# Autodesk Inventor assembly: ユニット4
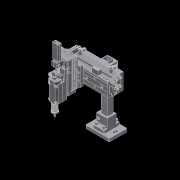
[picture p0: Inventor's stored thumbnail of the model, 180x180]
Saved by Autodesk Inventor 2021.1 (Build 251245010, 245A)
## iProperties
Created: 2008-11-13
Document SubType Name: Assembly
Title: ユニット4
## Documents named in this file (35)
- Z:\inventorroom\sample\unit4\unit4.iam
- Z:\inventorroom\sample\unit4\03.ipt
- Z:\inventorroom\sample\unit4\04.ipt
- Z:\inventorroom\sample\unit4\WSSM20-10-3.ipt
- Z:\inventorroom\sample\unit4\MHCAW10.ipt
- Z:\inventorroom\sample\unit4\07.ipt
- Z:\inventorroom\sample\unit4\AS1201F-M5-04.ipt
- Z:\inventorroom\sample\unit4\MXQ12-40AS\MXQ12-40AS-M9B.iam
- Z:\inventorroom\sample\unit4\MXQ16-75A\MXQ16-75A-M9B.iam
- Z:\inventorroom\sample\unit4\GT-H10.ipt
- Z:\inventorroom\sample\unit4\KJL06-M5.ipt
- Z:\inventorroom\sample\unit4\STAQ20-200.ipt
- Z:\inventorroom\sample\unit4\01.ipt
- Z:\inventorroom\sample\unit4\02.ipt
- Z:\inventorroom\sample\unit4\06.ipt
- Z:\inventorroom\sample\unit4\PSPWR10_100_M5_N6_SC10.ipt
- Z:\inventorroom\sample\unit4\SWU17_30.ipt
- Z:\inventorroom\sample\unit4\PSCKNK10-10\PSCKNK10-10.iam
- Z:\inventorroom\sample\unit4\05.ipt
- Z:\inventorroom\sample\unit4\CBM5_18.ipt
- Z:\inventorroom\sample\unit4\PWF5.ipt
- Z:\inventorroom\sample\unit4\SLW5.ipt
- Z:\inventorroom\sample\unit4\CLQAM20\CLQAM20.iam
- Z:\inventorroom\sample\unit4\CLTQAM20\CLTQAM20.iam
- Z:\inventorroom\sample\unit4\CBM5_30.ipt
- Z:\inventorroom\sample\unit4\CBM5_10.ipt
- Z:\inventorroom\sample\unit4\CBM4_20.ipt
- Z:\inventorroom\sample\unit4\CBM4_10.ipt
- Z:\inventorroom\sample\unit4\CBM4_6.ipt
- Z:\inventorroom\sample\unit4\CBM4_8.ipt
- Z:\inventorroom\sample\unit4\CBM4_15.ipt
- Z:\inventorroom\sample\unit4\MS5_10.ipt
- Z:\inventorroom\sample\unit4\MS4_10.ipt
- Z:\inventorroom\sample\unit4\worka.ipt
- Z:\inventorroom\sample\unit4\unit4\AIP\チューブ＆パイプ\unit4.チューブ＆パイプ配管.iam
## Components (73 placed, 34 different names)
1. 01:1 — 挿入:131, 挿入:132
2. 02:1 — 挿入:87, 挿入:88, 挿入:133, 挿入:134, 挿入:164, 挿入:165
3. 03:1 — 挿入:89, 挿入:90, 挿入:91, 挿入:92, 挿入:138, 挿入:139, 挿入:140, 挿入:141, 挿入:166, 挿入:167, 挿入:171, 挿入:172
4. 04:1 — 挿入:115, 挿入:116, 挿入:117, 挿入:118, 挿入:148, 挿入:149, 挿入:150, 挿入:151
5. 05:1 — 挿入:113, 挿入:114, 挿入:156, 挿入:157
6. 06:1 — 挿入:103, 挿入:108, 挿入:109, 角度:2, 挿入:145, 挿入:146, 挿入:147
7. 07:1 — 挿入:106, 挿入:170
8. MXQ16-75A-M9B:1 [sub-assembly] — 挿入:87, 挿入:88, 挿入:89, 挿入:90, 挿入:93, 挿入:94, 挿入:135, 挿入:136, 挿入:137
9. MXQ12-40AS-M9B:1 [sub-assembly] — 挿入:38, 挿入:39, 挿入:91, 挿入:92, 挿入:108, 挿入:109, 挿入:117, 挿入:118, 挿入:143, 挿入:144, 挿入:168, 挿入:169
10. AS1201F-M5-04:3 — 挿入:39
11. AS1201F-M5-04:4 — 挿入:38
12. AS1201F-M5-04:5 — 挿入:94
13. AS1201F-M5-04:6 — 挿入:93
14. KJL06-M5:1 — 挿入:105
15. GT-H10:1 — 挿入:103, 角度:2
16. PSCKNK10-10:1 [sub-assembly] — 挿入:112, 角度:1, メイト:137, 挿入:113, 挿入:114
17. MHCAW10:1 — 挿入:20, メイト:136, 角度:1, メイト:137, 挿入:115, 挿入:116, 挿入:152, 挿入:153, 挿入:154, 挿入:155
18. WSSM20-10-3:1 — 挿入:20
19. SWU17-30:1 — 挿入:107
20. PSPWR10-100-M5-N6-SC10:1 — 挿入:105, 挿入:106, 挿入:107, メイト:136, 挿入:112
21. CLQAM20:2 [sub-assembly] — 挿入:127, 挿入:128, 挿入:129, 挿入:130, 挿入:131, 挿入:132, メイト:138, メイト:139, フラッシュ:140
22. CLTQAM20:1 [sub-assembly] — メイト:140, メイト:141, フラッシュ:141, 挿入:133, 挿入:134, 挿入:162, 挿入:163
23. STAQ20-200:1 — メイト:138, メイト:139, フラッシュ:140, メイト:140, メイト:141, フラッシュ:141
24. CBM4-6:1 — 挿入:146
25. CBM4-6:2 — 挿入:147
26. CBM4-6:3 — 挿入:156
27. CBM4-6:4 — 挿入:157
28. CBM4-8:2 — 挿入:149
29. CBM4-8:1 — 挿入:148
30. CBM4-10:1 — 挿入:145
31. CBM4-15:1 — 挿入:150
32. CBM4-15:2 — 挿入:151
33. CBM4-20:2 — 挿入:143
34. CBM4-20:3 — 挿入:144
35. CBM4-20:4 — 挿入:152
36. CBM4-20:5 — 挿入:153
37. CBM4-20:6 — 挿入:154
38. CBM4-20:7 — 挿入:155
39. CBM5-10:1 — 挿入:138
40. CBM5-10:2 — 挿入:139
41. CBM5-10:3 — 挿入:140
42. CBM5-10:4 — 挿入:141
43. CBM5-18:1 — 挿入:119
44. CBM5-18:2 — 挿入:121
45. CBM5-18:3 — 挿入:123
46. CBM5-18:4 — 挿入:125
47. CBM5-18:5 — 挿入:161
48. CBM5-18:6 — 挿入:159
49. CBM5-30:1 — 挿入:135
50. CBM5-30:2 — 挿入:136
51. CBM5-30:3 — 挿入:137
52. SLW5:1 — 挿入:125, 挿入:126
53. SLW5:2 — 挿入:123, 挿入:124
54. SLW5:3 — 挿入:121, 挿入:122
55. SLW5:4 — 挿入:119, 挿入:120
56. SLW5:5 — 挿入:158, 挿入:159
57. SLW5:6 — 挿入:160, 挿入:161
58. PWF5:1 — 挿入:126, 挿入:128
59. PWF5:2 — 挿入:124, 挿入:127
60. PWF5:3 — 挿入:122, 挿入:129
61. PWF5:4 — 挿入:120, 挿入:130
62. PWF5:5 — 挿入:158, 挿入:162
63. PWF5:6 — 挿入:160, 挿入:163
64. MS4-10:1 — 挿入:166
65. MS4-10:2 — 挿入:167
66. MS4-10:3 — 挿入:168
67. MS4-10:4 — 挿入:169
68. MS5-10:1 — 挿入:165
69. MS5-10:2 — 挿入:164
70. worka:1 — 挿入:170
71. MS5-10:3 — 挿入:172
72. MS5-10:4 — 挿入:171
73. チューブ＆パイプ配管 [sub-assembly]
## Relationships (87: Insert 77, Mate 6, Angle 2, Flush 2)
- 挿入:20 [Insert]: MHCAW10:1 ↔ WSSM20-10-3:1
- 挿入:38 [Insert]: MXQ12-40AS-M9B:1 ↔ AS1201F-M5-04:4
- 挿入:39 [Insert]: MXQ12-40AS-M9B:1 ↔ AS1201F-M5-04:3
- 挿入:87 [Insert]: 02:1 ↔ MXQ16-75A-M9B:1
- 挿入:88 [Insert]: 02:1 ↔ MXQ16-75A-M9B:1
- 挿入:89 [Insert]: 03:1 ↔ MXQ16-75A-M9B:1
- 挿入:90 [Insert]: 03:1 ↔ MXQ16-75A-M9B:1
- 挿入:91 [Insert]: 03:1 ↔ MXQ12-40AS-M9B:1
- 挿入:92 [Insert]: 03:1 ↔ MXQ12-40AS-M9B:1
- 挿入:93 [Insert]: MXQ16-75A-M9B:1 ↔ AS1201F-M5-04:6
- 挿入:94 [Insert]: MXQ16-75A-M9B:1 ↔ AS1201F-M5-04:5
- 挿入:103 [Insert]: 06:1 ↔ GT-H10:1
- 挿入:105 [Insert]: KJL06-M5:1 ↔ PSPWR10-100-M5-N6-SC10:1
- 挿入:106 [Insert]: 07:1 ↔ PSPWR10-100-M5-N6-SC10:1
- 挿入:107 [Insert]: SWU17-30:1 ↔ PSPWR10-100-M5-N6-SC10:1
- 挿入:108 [Insert]: 06:1 ↔ MXQ12-40AS-M9B:1
- 挿入:109 [Insert]: 06:1 ↔ MXQ12-40AS-M9B:1
- メイト:136 [Mate]: MHCAW10:1 ↔ PSPWR10-100-M5-N6-SC10:1
- 挿入:112 [Insert] (6 mm): PSCKNK10-10:1 ↔ PSPWR10-100-M5-N6-SC10:1
- 角度:1 [Angle] (0 deg): PSCKNK10-10:1 ↔ MHCAW10:1
- メイト:137 [Mate]: PSCKNK10-10:1 ↔ MHCAW10:1
- 挿入:113 [Insert]: 05:1 ↔ PSCKNK10-10:1
- 挿入:114 [Insert]: 05:1 ↔ PSCKNK10-10:1
- 挿入:115 [Insert]: 04:1 ↔ MHCAW10:1
- 挿入:116 [Insert]: 04:1 ↔ MHCAW10:1
- 挿入:117 [Insert]: 04:1 ↔ MXQ12-40AS-M9B:1
- 挿入:118 [Insert]: 04:1 ↔ MXQ12-40AS-M9B:1
- 角度:2 [Angle] (0 deg): 06:1 ↔ GT-H10:1
- 挿入:119 [Insert]: CBM5-18:1 ↔ SLW5:4
- 挿入:120 [Insert]: SLW5:4 ↔ PWF5:4
- 挿入:121 [Insert]: CBM5-18:2 ↔ SLW5:3
- 挿入:122 [Insert]: SLW5:3 ↔ PWF5:3
- 挿入:123 [Insert]: CBM5-18:3 ↔ SLW5:2
- 挿入:124 [Insert]: SLW5:2 ↔ PWF5:2
- 挿入:125 [Insert]: CBM5-18:4 ↔ SLW5:1
- 挿入:126 [Insert]: SLW5:1 ↔ PWF5:1
- 挿入:127 [Insert]: CLQAM20:2 ↔ PWF5:2
- 挿入:128 [Insert]: CLQAM20:2 ↔ PWF5:1
- 挿入:129 [Insert]: CLQAM20:2 ↔ PWF5:3
- 挿入:130 [Insert]: CLQAM20:2 ↔ PWF5:4
- 挿入:131 [Insert]: 01:1 ↔ CLQAM20:2
- 挿入:132 [Insert]: 01:1 ↔ CLQAM20:2
- メイト:138 [Mate]: CLQAM20:2 ↔ STAQ20-200:1
- メイト:139 [Mate]: CLQAM20:2 ↔ STAQ20-200:1
- フラッシュ:140 [Flush]: CLQAM20:2 ↔ STAQ20-200:1
- メイト:140 [Mate]: CLTQAM20:1 ↔ STAQ20-200:1
- メイト:141 [Mate]: CLTQAM20:1 ↔ STAQ20-200:1
- フラッシュ:141 [Flush] (10 mm): CLTQAM20:1 ↔ STAQ20-200:1
- 挿入:133 [Insert]: 02:1 ↔ CLTQAM20:1
- 挿入:134 [Insert]: 02:1 ↔ CLTQAM20:1
- 挿入:135 [Insert]: MXQ16-75A-M9B:1 ↔ CBM5-30:1
- 挿入:136 [Insert]: MXQ16-75A-M9B:1 ↔ CBM5-30:2
- 挿入:137 [Insert]: MXQ16-75A-M9B:1 ↔ CBM5-30:3
- 挿入:138 [Insert]: 03:1 ↔ CBM5-10:1
- 挿入:139 [Insert]: 03:1 ↔ CBM5-10:2
- 挿入:140 [Insert]: 03:1 ↔ CBM5-10:3
- 挿入:141 [Insert]: 03:1 ↔ CBM5-10:4
- 挿入:143 [Insert]: MXQ12-40AS-M9B:1 ↔ CBM4-20:2
- 挿入:144 [Insert]: MXQ12-40AS-M9B:1 ↔ CBM4-20:3
- 挿入:145 [Insert]: 06:1 ↔ CBM4-10:1
- 挿入:146 [Insert]: 06:1 ↔ CBM4-6:1
- 挿入:147 [Insert]: 06:1 ↔ CBM4-6:2
- 挿入:148 [Insert]: 04:1 ↔ CBM4-8:1
- 挿入:149 [Insert]: 04:1 ↔ CBM4-8:2
- 挿入:150 [Insert]: 04:1 ↔ CBM4-15:1
- 挿入:151 [Insert]: 04:1 ↔ CBM4-15:2
- 挿入:152 [Insert]: MHCAW10:1 ↔ CBM4-20:4
- 挿入:153 [Insert]: MHCAW10:1 ↔ CBM4-20:5
- 挿入:154 [Insert]: MHCAW10:1 ↔ CBM4-20:6
- 挿入:155 [Insert]: MHCAW10:1 ↔ CBM4-20:7
- 挿入:156 [Insert]: 05:1 ↔ CBM4-6:3
- 挿入:157 [Insert]: 05:1 ↔ CBM4-6:4
- 挿入:158 [Insert]: SLW5:5 ↔ PWF5:5
- 挿入:159 [Insert]: CBM5-18:6 ↔ SLW5:5
- 挿入:160 [Insert]: SLW5:6 ↔ PWF5:6
- 挿入:161 [Insert]: CBM5-18:5 ↔ SLW5:6
- 挿入:162 [Insert]: CLTQAM20:1 ↔ PWF5:5
- 挿入:163 [Insert]: CLTQAM20:1 ↔ PWF5:6
- 挿入:164 [Insert] (2 mm): 02:1 ↔ MS5-10:2
- 挿入:165 [Insert] (2 mm): 02:1 ↔ MS5-10:1
- 挿入:166 [Insert] (2 mm): 03:1 ↔ MS4-10:1
- 挿入:167 [Insert] (2 mm): 03:1 ↔ MS4-10:2
- 挿入:168 [Insert] (2 mm): MXQ12-40AS-M9B:1 ↔ MS4-10:3
- 挿入:169 [Insert] (2 mm): MXQ12-40AS-M9B:1 ↔ MS4-10:4
- 挿入:170 [Insert]: 07:1 ↔ worka:1
- 挿入:171 [Insert] (2 mm): 03:1 ↔ MS5-10:4
- 挿入:172 [Insert] (2 mm): 03:1 ↔ MS5-10:3
